# Autodesk Inventor assembly: CNC-Y-axis- ASSEMBLYg
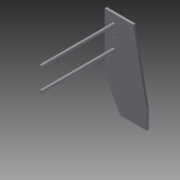
[picture p0: Inventor's stored thumbnail of the model, 180x180]
Saved by Autodesk Inventor 2015 (Build 190159000, 159)
## iProperties
Created: 2015-03-24
Part Number: CNC-Y-axis- ASSEMBLYg
Document SubType Name: Assembly
Designer: Bangladesh
Author: Bangladesh
## Documents named in this file (3)
- C:\Users\Alvi\Documents\CNC design files\Assemblies\CNC-Y-axis- ASSEMBLY.iam
- C:\Users\Alvi\Documents\CNC design files\CNC-Y-axis- side plates.ipt
- C:\Users\Alvi\Documents\CNC design files\CNC-Y-axs- sliding rod.ipt
## Components (3 placed, 2 different names)
1. CNC-Y-axis- side plates:1 — Mate:1, Mate:2
2. CNC-Y-axs- sliding rod:1 — Mate:1
3. CNC-Y-axs- sliding rod:2 — Mate:2
## Relationships (2: Mate 2)
- Mate:1: CNC-Y-axis- side plates:1 ↔ CNC-Y-axs- sliding rod:1
- Mate:2: CNC-Y-axis- side plates:1 ↔ CNC-Y-axs- sliding rod:2
